# Autodesk Inventor assembly: 45degreebracketassembly
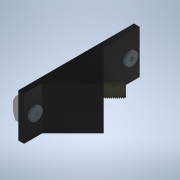
[picture p0: Inventor's stored thumbnail of the model, 180x180]
Saved by Autodesk Inventor 2020.2 (Build 242310000, 310)
## iProperties
Created: 2020-07-25
Part Number: 45degreebracketassembly
Document SubType Name: Assembly
Designer: JK
Author: JK
## Documents named in this file (5)
- C:\Users\JK\Documents\Inventor\Mesa\45degreebracketassembly.iam
- C:\Users\JK\Documents\Inventor\Mesa\45degreebracket.ipt
- C:\Users\JK\Documents\Inventor\Mesa\M5x12BoltFlatHead.ipt
- C:\Users\JK\Documents\Inventor\Mesa\T_Slot_Nut_Dropin_3030m5ipt.ipt
- C:\Users\JK\Documents\Inventor\Mesa\M8x16socketheadbolt.ipt
## Components (6 placed, 4 different names)
1. 45degreebracket:1 — Mate:1, Mate:2, Angle:1, Mate:4, Mate:5, Mate:6, Angle:2, Mate:8, Mate:9, Mate:10
2. M5x12BoltFlatHead:1 — Mate:1, Mate:2, Mate:3
3. M5x12BoltFlatHead:2 — Mate:5, Mate:6, Mate:7
4. T_Slot_Nut_Dropin_3030m5ipt:1 — Mate:3, Angle:1, Mate:4
5. T_Slot_Nut_Dropin_3030m5ipt:2 — Mate:7, Angle:2, Mate:8
6. M8x16socketheadbolt:1 — Mate:9, Mate:10
## Relationships (12: Mate 10, Angle 2)
- Mate:1: 45degreebracket:1 ↔ M5x12BoltFlatHead:1
- Mate:2: 45degreebracket:1 ↔ M5x12BoltFlatHead:1
- Mate:3: M5x12BoltFlatHead:1 ↔ T_Slot_Nut_Dropin_3030m5ipt:1
- Angle:1 (0 deg): 45degreebracket:1 ↔ T_Slot_Nut_Dropin_3030m5ipt:1
- Mate:4: 45degreebracket:1 ↔ T_Slot_Nut_Dropin_3030m5ipt:1
- Mate:5: 45degreebracket:1 ↔ M5x12BoltFlatHead:2
- Mate:6: 45degreebracket:1 ↔ M5x12BoltFlatHead:2
- Mate:7: M5x12BoltFlatHead:2 ↔ T_Slot_Nut_Dropin_3030m5ipt:2
- Angle:2 (0 deg): 45degreebracket:1 ↔ T_Slot_Nut_Dropin_3030m5ipt:2
- Mate:8: 45degreebracket:1 ↔ T_Slot_Nut_Dropin_3030m5ipt:2
- Mate:9: 45degreebracket:1 ↔ M8x16socketheadbolt:1
- Mate:10: 45degreebracket:1 ↔ M8x16socketheadbolt:1
